# Autodesk Inventor assembly: 3.25'' Omni-Directional Wheel, Free Spinning Insert
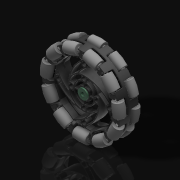
[picture p0: Inventor's stored thumbnail of the model, 180x180]
Saved by Autodesk Inventor 2021 (Build 250183000, 183)
## iProperties
Created: 2014-06-25
Document SubType Name: Assembly
Designer: Jordan Kiesel
Vendor: VEX Robotics, Inc.
Mass: 62.3747 g
Surface Area: 582.757 cm^2
Volume: 43.4615 cm^3
Part Number: 3.25'' Omni-Directional Wheel, Free Spinning Insert
Density: 1.43517 g/cm^3
Company: Bots 'n' Stuff
Author: Jordan Kiesel
Title: 3.25" Omni-Directional Wheel, Square Insert
## Documents named in this file (3)
- E:\VEX Library\Motion\Wheels _ Rollers\3.25 Omni, Free Spinning Insert.iam
- E:\VEX Library\Motion\Wheels _ Rollers\Reference Parts\3.25_ Omni-Directional Wheels\3.25_ Omni-Directional Wheel.iam
- E:\VEX Library\Motion\Reference Parts\Free Spinning Gear Insert.ipt
## Components (3 placed, 2 different names)
1. 3.25_ Omni-Directional Wheel:1 [sub-assembly] — Mate:3, Mate:6
2. Free Spinning Gear Insert:1 — Mate:3
3. Free Spinning Gear Insert:2 — Mate:6
## Relationships (6: Mate 6)
- [Mate] (0.0254 mm): 3.25_ Omni-Directional Wheel:1 ↔ Free Spinning Gear Insert:1
- [Mate] (0.0254 mm): 3.25_ Omni-Directional Wheel:1 ↔ Free Spinning Gear Insert:1
- Mate:3: 3.25_ Omni-Directional Wheel:1 ↔ Free Spinning Gear Insert:1
- [Mate] (0.0254 mm): 3.25_ Omni-Directional Wheel:1 ↔ Free Spinning Gear Insert:2
- [Mate] (0.0254 mm): 3.25_ Omni-Directional Wheel:1 ↔ Free Spinning Gear Insert:2
- Mate:6: 3.25_ Omni-Directional Wheel:1 ↔ Free Spinning Gear Insert:2
